# Autodesk Inventor assembly: GGC
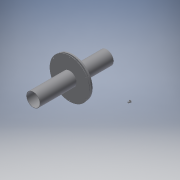
[picture p0: Inventor's stored thumbnail of the model, 180x180]
Saved by Autodesk Inventor 2016 (Build 200138000, 138)
## iProperties
Created: 2016-04-11
Part Number: GGC
Document SubType Name: Assembly
Designer: rubenjm
Author: rubenjm
## Documents named in this file (6)
- C:\Users\rmarkowi\Documents\GGC\GGC.iam
- C:\Users\rmarkowi\Documents\GGC\Inner Pole.ipt
- C:\Users\rmarkowi\Documents\GGC\Base Plate.ipt
- C:\Users\rmarkowi\Documents\GGC\Turntable_2.ipt
- C:\Users\rmarkowi\Documents\GGC\Top Plate.ipt
- C:\Users\rmarkowi\Documents\GGC\Small Gear.ipt
## Components (6 placed, 5 different names)
1. Inner Pole:1 — Flush:1, Mate:2, Mate:3, Cylindrical:1
2. Base Plate:1 — Flush:1, Mate:1, Mate:3, Mate:4
3. Turntable_2:1 — Mate:1, Mate:2, Mate:4, Mate:7
4. Top Plate:1 — Mate:6, Tangent:1, Tangent:2, Mate:7
5. Top Plate:2 — Mate:6, Tangent:1, Tangent:2, Cylindrical:1
6. Small Gear:1
## Relationships (10: Mate 6, Tangent 2, Flush 1, CylindricalJoint 1)
- Flush:1 (304.8 mm): Inner Pole:1 ↔ Base Plate:1
- Mate:1 (12.7 mm): Base Plate:1 ↔ Turntable_2:1
- Mate:2: Inner Pole:1 ↔ Turntable_2:1
- Mate:3: Inner Pole:1 ↔ Base Plate:1
- Mate:4: Base Plate:1 ↔ Turntable_2:1
- Mate:6: Top Plate:1 ↔ Top Plate:2
- Tangent:1: Top Plate:1 ↔ Top Plate:2
- Tangent:2: Top Plate:1 ↔ Top Plate:2
- Cylindrical:1: Inner Pole:1 ↔ Top Plate:2
- Mate:7: Turntable_2:1 ↔ Top Plate:1
